# Autodesk Inventor assembly: Top
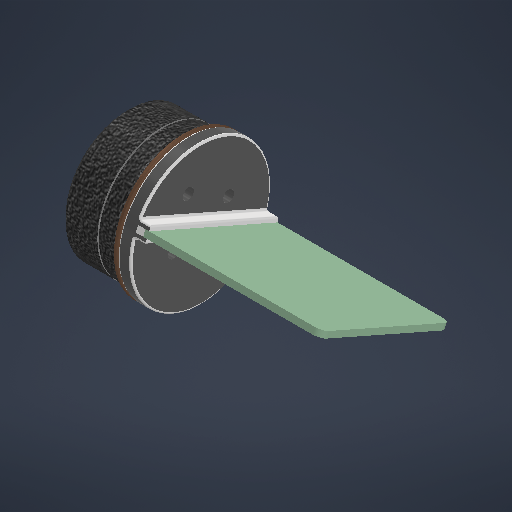
[picture p0: Inventor's stored thumbnail of the model, 512x512]
Saved by Autodesk Inventor 2026.1 (Build 301233020, 233B)
## iProperties
Created: 2026-05-23
Part Number: Top
Document SubType Name: Assembly
Designer: InventorKid
Author: InventorKid
## Documents named in this file (5)
- C:\Users\InventorKid\Documents\Volumetric Display\Top.iam
- C:\Users\InventorKid\Documents\Volumetric Display\Motor.ipt
- C:\Users\InventorKid\Documents\Volumetric Display\Stand.ipt
- C:\Users\InventorKid\Documents\Volumetric Display\Coil.ipt
- C:\Users\InventorKid\Documents\Volumetric Display\PCB.ipt
## Components (4 placed, 4 different names)
1. Motor:1 — Mate:1, Insert:2, Insert:3
2. Stand:1 — Mate:1, Mate:2, Insert:1, Insert:2, Insert:3, Mate:3, Mate:4, Mate:5
3. Coil:1 — Mate:2, Insert:1
4. PCB:1 — Mate:3, Mate:4, Mate:5
## Relationships (8: Mate 5, Insert 3)
- Mate:1 (0.2 mm): Motor:1 ↔ Stand:1
- Mate:2 (0.05 mm): Stand:1 ↔ Coil:1
- Insert:1 (0.05 mm): Stand:1 ↔ Coil:1
- Insert:2 (0.2 mm): Motor:1 ↔ Stand:1
- Insert:3 (0.2 mm): Motor:1 ↔ Stand:1
- Mate:3: Stand:1 ↔ PCB:1
- Mate:4: Stand:1 ↔ PCB:1
- Mate:5: Stand:1 ↔ PCB:1
## Named parameters: Finish1_Area = 12.1728, Finish2_Area = 33.3326, Finish3_Area = 28.5173
note: some values were not read from the file. Shown as the stored number, unit unknown: "Finish1_Area", "Finish2_Area", "Finish3_Area".
